# Autodesk Inventor assembly: TT_Intake
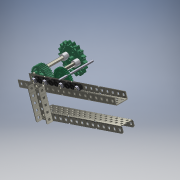
[picture p0: Inventor's stored thumbnail of the model, 180x180]
Saved by Autodesk Inventor 2019 (Build 230136000, 136)
## iProperties
Created: 2020-02-10
Part Number: TT_Intake
Document SubType Name: Assembly
Designer: clove
Author: clove
## Documents named in this file (18)
- C:\Users\clove\Downloads\TT_Intake.iam
- C:\Users\clove\Downloads\SID Library-20181221T040531Z-001\2018 BNS-VRC-SID Library\Structure\C-Channels\C-Channel 1x2x1\Aluminum C-Channel 1x2x1x18.ipt
- C:\Users\clove\Downloads\SID Library-20181221T040531Z-001\2018 BNS-VRC-SID Library\Structure\C-Channels\C-Channel 1x2x1\Aluminum C-Channel 1x2x1x15.ipt
- C:\Users\clove\Downloads\SID Library-20181221T040531Z-001\2018 BNS-VRC-SID Library\Structure\C-Channels\C-Channel 1x2x1\Aluminum C-Channel 1x2x1x5.ipt
- C:\Users\clove\Downloads\SID Library-20181221T040531Z-001\2018 BNS-VRC-SID Library\Structure\Screws _ Nuts\Screw 8-32 x 0.375_.ipt
- C:\Users\clove\Downloads\SID Library-20181221T040531Z-001\2018 BNS-VRC-SID Library\Structure\Screws _ Nuts\8-32 Nylon-Insert Thin Hex Locknut.iam
- C:\Users\clove\Downloads\SID Library-20181221T040531Z-001\2018 BNS-VRC-SID Library\Motion\Bearing Flat.ipt
- C:\Users\clove\Downloads\SID Library-20181221T040531Z-001\2018 BNS-VRC-SID Library\Structure\Screws _ Nuts\Screw 8-32 x 0.500_.ipt
- C:\Users\clove\Downloads\SID Library-20181221T040531Z-001\2018 BNS-VRC-SID Library\Motion\Spur Gears\High Strength 36-tooth Gear-Free Spinning Insert.iam
- C:\Users\clove\Downloads\SID Library-20181221T040531Z-001\2018 BNS-VRC-SID Library\Motion\Washers _ Spacers\Spacer (Nylon), 0.125_.ipt
- C:\Users\clove\Downloads\SID Library-20181221T040531Z-001\2018 BNS-VRC-SID Library\Structure\Screws _ Nuts\Nut 8-32 Keps.ipt
- C:\Users\clove\Downloads\SID Library-20181221T040531Z-001\2018 BNS-VRC-SID Library\Structure\Screws _ Nuts\Screw 8-32 x 1.250_.ipt
- C:\Users\clove\Downloads\SID Library-20181221T040531Z-001\2018 BNS-VRC-SID Library\Structure\Screws _ Nuts\Screw 8-32 x 0.875_.ipt
- C:\Users\clove\Downloads\SID Library-20181221T040531Z-001\2018 BNS-VRC-SID Library\Structure\Standoffs _ Couplers\Standoff 2.00_.ipt
- C:\Users\clove\Downloads\SID Library-20181221T040531Z-001\2018 BNS-VRC-SID Library\Motion\Washers _ Spacers\Spacer (Nylon), 0.375_.ipt
- C:\Users\clove\Downloads\SID Library-20181221T040531Z-001\2018 BNS-VRC-SID Library\Motion\Sprockets\High Strength 18-tooth Sprocket.ipt
- C:\Users\clove\Downloads\SID Library-20181221T040531Z-001\2018 BNS-VRC-SID Library\Motion\Spur Gears\36-tooth Gear.ipt
- C:\Users\clove\Downloads\SID Library-20181221T040531Z-001\2018 BNS-VRC-SID Library\Motion\Drive Shafts\Drive Shaft 3_.ipt
## Components (34 placed, 17 different names)
1. Aluminum C-Channel 1x2x1x18:1 — Insert:3, Insert:4, Insert:9, Insert:10, Insert:15, Insert:16, Insert:17, Insert:18, Insert:19, Insert:20, Insert:21, Insert:22, Insert:24, Insert:26, Insert:30
2. Aluminum C-Channel 1x2x1x15:1 — Insert:1, Insert:2, Insert:11, Insert:12
3. Aluminum C-Channel 1x2x1x5:1 — Insert:1, Insert:2, Insert:3, Insert:4, Insert:5, Insert:6, Insert:7, Insert:8
4. Screw 8-32 x 0.375_:1 — Insert:5
5. Screw 8-32 x 0.375_:2 — Insert:6
6. Screw 8-32 x 0.375_:3 — Insert:7
7. Screw 8-32 x 0.375_:4 — Insert:8
8. 8-32 Nylon-Insert Thin Hex Locknut:1 [sub-assembly] — Insert:9
9. 8-32 Nylon-Insert Thin Hex Locknut:2 [sub-assembly] — Insert:10
10. 8-32 Nylon-Insert Thin Hex Locknut:3 [sub-assembly] — Insert:11
11. 8-32 Nylon-Insert Thin Hex Locknut:4 [sub-assembly] — Insert:12
12. Bearing Flat:2 — Insert:15, Insert:16, Insert:25
13. Bearing Flat:3 — Insert:17, Insert:18, Insert:19, Insert:27
14. Bearing Flat:4 — Insert:20, Insert:21, Insert:23, Insert:33
15. Screw 8-32 x 0.500_:1 — Insert:22
16. 8-32 Nylon-Insert Thin Hex Locknut:5 [sub-assembly] — Insert:23
17. Screw 8-32 x 0.500_:2 — Insert:24
18. 8-32 Nylon-Insert Thin Hex Locknut:6 [sub-assembly] — Insert:33
19. 8-32 Nylon-Insert Thin Hex Locknut:7 [sub-assembly] — Insert:25
20. Screw 8-32 x 0.500_:3 — Insert:26
21. 8-32 Nylon-Insert Thin Hex Locknut:8 [sub-assembly] — Insert:27
22. High Strength 36-tooth Gear-Free Spinning Insert:1 [sub-assembly] — Insert:28, Insert:31, Insert:34, Insert:35, Insert:36, Insert:37
23. Spacer (Nylon), 0.125_:1 — Insert:28, Insert:32
24. Nut 8-32 Keps:1 — Insert:30, Insert:31
25. Screw 8-32 x 1.250_:1 — Insert:32
26. Screw 8-32 x 0.875_:1 — Insert:34
27. Screw 8-32 x 0.875_:2 — Insert:35
28. Standoff 2.00_:1 — Insert:36, Insert:38
29. Standoff 2.00_:2 — Insert:37, Insert:39
30. Spacer (Nylon), 0.375_:1 — Insert:38, Insert:41
31. Spacer (Nylon), 0.375_:2 — Insert:39, Insert:40
32. High Strength 18-tooth Sprocket:1 — Insert:40, Insert:41
33. 36-tooth Gear:1
34. Drive Shaft 3_:1
## Relationships (38: Insert 38)
- Insert:1: Aluminum C-Channel 1x2x1x15:1 ↔ Aluminum C-Channel 1x2x1x5:1
- Insert:2: Aluminum C-Channel 1x2x1x15:1 ↔ Aluminum C-Channel 1x2x1x5:1
- Insert:3: Aluminum C-Channel 1x2x1x18:1 ↔ Aluminum C-Channel 1x2x1x5:1
- Insert:4: Aluminum C-Channel 1x2x1x18:1 ↔ Aluminum C-Channel 1x2x1x5:1
- Insert:5: Aluminum C-Channel 1x2x1x5:1 ↔ Screw 8-32 x 0.375_:1
- Insert:6: Aluminum C-Channel 1x2x1x5:1 ↔ Screw 8-32 x 0.375_:2
- Insert:7: Aluminum C-Channel 1x2x1x5:1 ↔ Screw 8-32 x 0.375_:3
- Insert:8: Aluminum C-Channel 1x2x1x5:1 ↔ Screw 8-32 x 0.375_:4
- Insert:9: Aluminum C-Channel 1x2x1x18:1 ↔ 8-32 Nylon-Insert Thin Hex Locknut:1
- Insert:10: Aluminum C-Channel 1x2x1x18:1 ↔ 8-32 Nylon-Insert Thin Hex Locknut:2
- Insert:11: Aluminum C-Channel 1x2x1x15:1 ↔ 8-32 Nylon-Insert Thin Hex Locknut:3
- Insert:12: Aluminum C-Channel 1x2x1x15:1 ↔ 8-32 Nylon-Insert Thin Hex Locknut:4
- Insert:15: Aluminum C-Channel 1x2x1x18:1 ↔ Bearing Flat:2
- Insert:16: Aluminum C-Channel 1x2x1x18:1 ↔ Bearing Flat:2
- Insert:17: Aluminum C-Channel 1x2x1x18:1 ↔ Bearing Flat:3
- Insert:18: Aluminum C-Channel 1x2x1x18:1 ↔ Bearing Flat:3
- Insert:19: Aluminum C-Channel 1x2x1x18:1 ↔ Bearing Flat:3
- Insert:20: Aluminum C-Channel 1x2x1x18:1 ↔ Bearing Flat:4
- Insert:21: Aluminum C-Channel 1x2x1x18:1 ↔ Bearing Flat:4
- Insert:22: Aluminum C-Channel 1x2x1x18:1 ↔ Screw 8-32 x 0.500_:1
- Insert:23: Bearing Flat:4 ↔ 8-32 Nylon-Insert Thin Hex Locknut:5
- Insert:24: Aluminum C-Channel 1x2x1x18:1 ↔ Screw 8-32 x 0.500_:2
- Insert:25: Bearing Flat:2 ↔ 8-32 Nylon-Insert Thin Hex Locknut:7
- Insert:26: Aluminum C-Channel 1x2x1x18:1 ↔ Screw 8-32 x 0.500_:3
- Insert:27: Bearing Flat:3 ↔ 8-32 Nylon-Insert Thin Hex Locknut:8
- Insert:28: High Strength 36-tooth Gear-Free Spinning Insert:1 ↔ Spacer (Nylon), 0.125_:1
- Insert:30: Aluminum C-Channel 1x2x1x18:1 ↔ Nut 8-32 Keps:1
- Insert:31: High Strength 36-tooth Gear-Free Spinning Insert:1 ↔ Nut 8-32 Keps:1
- Insert:32: Spacer (Nylon), 0.125_:1 ↔ Screw 8-32 x 1.250_:1
- Insert:33: Bearing Flat:4 ↔ 8-32 Nylon-Insert Thin Hex Locknut:6
- Insert:34: High Strength 36-tooth Gear-Free Spinning Insert:1 ↔ Screw 8-32 x 0.875_:1
- Insert:35: High Strength 36-tooth Gear-Free Spinning Insert:1 ↔ Screw 8-32 x 0.875_:2
- Insert:36: High Strength 36-tooth Gear-Free Spinning Insert:1 ↔ Standoff 2.00_:1
- Insert:37: High Strength 36-tooth Gear-Free Spinning Insert:1 ↔ Standoff 2.00_:2
- Insert:38: Standoff 2.00_:1 ↔ Spacer (Nylon), 0.375_:1
- Insert:39: Standoff 2.00_:2 ↔ Spacer (Nylon), 0.375_:2
- Insert:40: Spacer (Nylon), 0.375_:2 ↔ High Strength 18-tooth Sprocket:1
- Insert:41: Spacer (Nylon), 0.375_:1 ↔ High Strength 18-tooth Sprocket:1
